# Autodesk Inventor assembly: motor_spool
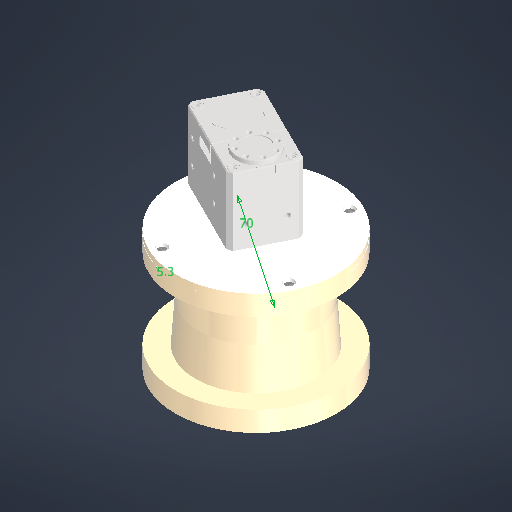
[picture p0: Inventor's stored thumbnail of the model, 512x512]
Saved by Autodesk Inventor 2026.2 (Build 302298010, 298A)
## iProperties
Created: 2026-03-01
Part Number: motor_spool
Document SubType Name: Assembly
Designer: Luke
Author: Luke
## Documents named in this file (3)
- C:\Users\Luke\OneDrive - Heriot-Watt University\Desktop\Robot Mech Sys\GroupProject\CAD\sub_assemblies\motor_spool_sub_assem.iam
- C:\Users\Luke\OneDrive - Heriot-Watt University\Desktop\Robot Mech Sys\GroupProject\CAD\parts\motor_imported_Simplify_1.ipt
- C:\Users\Luke\OneDrive - Heriot-Watt University\Desktop\Robot Mech Sys\GroupProject\CAD\sub_assemblies\spool_sub_assem.iam
## Components (2 placed, 2 different names)
1. spool_sub_assem:1 [sub-assembly] — Mate:1, Mate:2, Mate:3
2. motor_imported_Simplify_1:1 — Mate:1, Mate:3
## Relationships (3: Mate 3)
- Mate:1: spool_sub_assem:1 ↔ motor_imported_Simplify_1:1
- Mate:2: spool_sub_assem:1
- Mate:3: spool_sub_assem:1 ↔ motor_imported_Simplify_1:1
